# Autodesk Inventor assembly: 10mm_cnc_v1
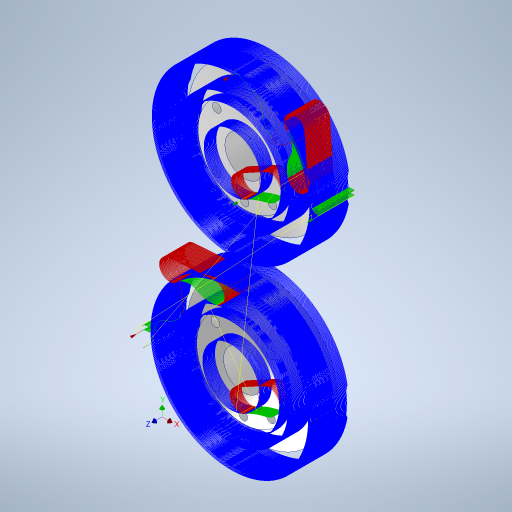
[picture p0: Inventor's stored thumbnail of the model, 512x512]
Saved by Autodesk Inventor 2024.3 (Build 283343010, 343A)
## iProperties
Created: 2025-07-12
Part Number: 10mm_cnc_v1
Document SubType Name: Assembly
Designer: tanoue_kota
Author: tanoue_kota
## Documents named in this file (2)
- C:\Users\kshau\Documents\inventor\Create_ViperX\Create_ViperX_ALOHA\FlatPattern\10mm_cnc_v1.iam
- C:\Users\kshau\Documents\inventor\Create_ViperX\Create_ViperX_ALOHA\ForeArm_Component\connectplate5.ipt
## Components (2 placed, 1 different names)
1. connectplate5:1 — フラッシュ:1
2. connectplate5:2 — フラッシュ:1
## Relationships (1: Flush 1)
- フラッシュ:1 [Flush]: connectplate5:1 ↔ connectplate5:2
